# Autodesk Inventor assembly: brush end effector
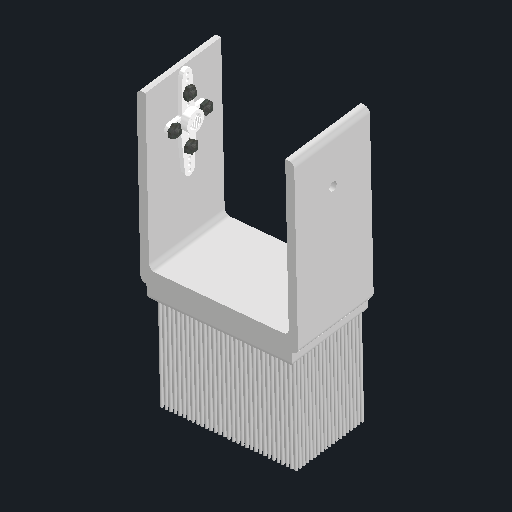
[picture p0: Inventor's stored thumbnail of the model, 512x512]
Saved by Autodesk Inventor 2024.2 (Build 282272000, 272)
## iProperties
Created: 2024-03-20
Part Number: brush end effector
Document SubType Name: Assembly
Designer: seifs
Author: seifs
## Documents named in this file (5)
- C:\Users\seifs\Downloads\Final Assembly\brush end effector_3.iam
- C:\Users\seifs\Downloads\Final Assembly\SG90 - Micro Servo 9g - Tower Pro.4.ipt
- C:\Users\seifs\Downloads\Final Assembly\final brush.ipt
- C:\Users\seifs\OneDrive\Documents\Inventor\Content Center Files\R2024\en-US\ISO 7046-1 Z(1)\ISO 7046-1 - M2 x 8_ - 4.8 - Z - ISO.ipt
- C:\Users\seifs\OneDrive\Documents\Inventor\Content Center Files\R2024\en-US\ISO 4036(2)\ISO 4036 - M2(2).ipt
## Components (10 placed, 4 different names)
1. SG90 - Micro Servo 9g - Tower Pro.4:2 — Insert:9, Insert:10, Mate:5, Mate:7, Mate:9, Mate:11
2. final brush:1 — Insert:9, Insert:10, Insert:26, Insert:27, Insert:28, Insert:29
3. ISO 7046-1 Z M2 x 8 - 4.8 - Z:4 — Insert:28, Mate:8
4. ISO 7046-1 Z M2 x 8 - 4.8 - Z:5 — Insert:27, Mate:4
5. ISO 7046-1 Z M2 x 8 - 4.8 - Z:6 — Insert:29, Mate:10
6. ISO 7046-1 Z M2 x 8 - 4.8 - Z:7 — Insert:26, Mate:6
7. ISO 4036 M2:4 — Mate:4, Mate:5
8. ISO 4036 M2:5 — Mate:8, Mate:9
9. ISO 4036 M2:6 — Mate:6, Mate:7
10. ISO 4036 M2:7 — Mate:10, Mate:11
## Relationships (14: Mate 8, Insert 6)
- Insert:9: SG90 - Micro Servo 9g - Tower Pro.4:2 ↔ final brush:1
- Insert:10: SG90 - Micro Servo 9g - Tower Pro.4:2 ↔ final brush:1
- Insert:26: final brush:1 ↔ ISO 7046-1 Z M2 x 8 - 4.8 - Z:7
- Insert:27: final brush:1 ↔ ISO 7046-1 Z M2 x 8 - 4.8 - Z:5
- Insert:28: final brush:1 ↔ ISO 7046-1 Z M2 x 8 - 4.8 - Z:4
- Insert:29: final brush:1 ↔ ISO 7046-1 Z M2 x 8 - 4.8 - Z:6
- Mate:4: ISO 7046-1 Z M2 x 8 - 4.8 - Z:5 ↔ ISO 4036 M2:4
- Mate:5: SG90 - Micro Servo 9g - Tower Pro.4:2 ↔ ISO 4036 M2:4
- Mate:6: ISO 7046-1 Z M2 x 8 - 4.8 - Z:7 ↔ ISO 4036 M2:6
- Mate:7: SG90 - Micro Servo 9g - Tower Pro.4:2 ↔ ISO 4036 M2:6
- Mate:8: ISO 7046-1 Z M2 x 8 - 4.8 - Z:4 ↔ ISO 4036 M2:5
- Mate:9: SG90 - Micro Servo 9g - Tower Pro.4:2 ↔ ISO 4036 M2:5
- Mate:10: ISO 7046-1 Z M2 x 8 - 4.8 - Z:6 ↔ ISO 4036 M2:7
- Mate:11: SG90 - Micro Servo 9g - Tower Pro.4:2 ↔ ISO 4036 M2:7
